# Autodesk Inventor assembly: CaseC
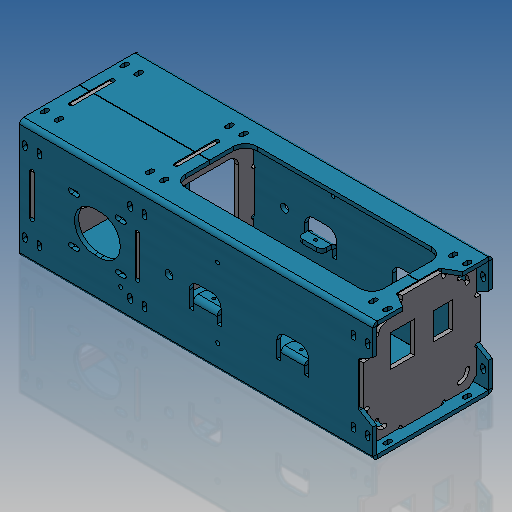
[picture p0: Inventor's stored thumbnail of the model, 512x512]
Saved by Autodesk Inventor 2017 (Build 210142000, 142)
## iProperties
Part Number: CaseC
Material: Genérico
Document SubType Name: Assembly
Designer: Leo
Author: Leo
## Documents named in this file (6)
- C:\Users\Leo\Documents\GitHub\actor-re-actor\models\inventor-caja\CaseC.iam
- C:\Users\Leo\Documents\GitHub\actor-re-actor\models\inventor-caja\Case\Protector.ipt
- C:\Users\Leo\Documents\GitHub\actor-re-actor\models\inventor-caja\Case\Pieza4.ipt
- C:\Users\Leo\Documents\GitHub\actor-re-actor\models\inventor-caja\Case\Pliegue Principal.ipt
- C:\Users\Leo\Documents\GitHub\actor-re-actor\models\inventor-caja\Case\refuerzo interior.ipt
- C:\Users\Leo\Documents\GitHub\actor-re-actor\models\inventor-caja\Case\Tapa Enchufes b.ipt
## Components (5 placed, 5 different names)
1. Pliegue Principal:1 — Nivelación:8, Nivelación:10, Nivelación:11, Nivelación:13, Nivelación:15, Coincidencia:3
2. Protector:1 — Nivelación:1, Nivelación:2, Nivelación:3
3. Tapa Enchufes b:1 — Nivelación:8, Nivelación:9, Nivelación:10
4. Pieza4:1 — Nivelación:11, Nivelación:12, Nivelación:13
5. refuerzo interior:1 — Nivelación:14, Nivelación:15, Coincidencia:3
## Relationships (12: Flush 11, Mate 1)
- Nivelación:1 [Flush] (40 mm): Protector:1
- Nivelación:2 [Flush]: Protector:1
- Nivelación:3 [Flush]: Protector:1
- Nivelación:8 [Flush]: Pliegue Principal:1 ↔ Tapa Enchufes b:1
- Nivelación:9 [Flush]: Tapa Enchufes b:1
- Nivelación:10 [Flush]: Pliegue Principal:1 ↔ Tapa Enchufes b:1
- Nivelación:11 [Flush]: Pliegue Principal:1 ↔ Pieza4:1
- Nivelación:12 [Flush]: Pieza4:1
- Nivelación:13 [Flush]: Pliegue Principal:1 ↔ Pieza4:1
- Nivelación:14 [Flush]: refuerzo interior:1
- Nivelación:15 [Flush]: Pliegue Principal:1 ↔ refuerzo interior:1
- Coincidencia:3 [Mate]: Pliegue Principal:1 ↔ refuerzo interior:1
